# Autodesk Inventor assembly: ARM1
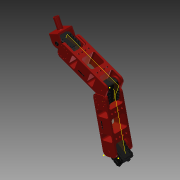
[picture p0: Inventor's stored thumbnail of the model, 180x180]
Saved by Autodesk Inventor 2015 (Build 190159000, 159)
## iProperties
Created: 2016-12-02
Part Number: ARM1
Document SubType Name: Assembly
Designer: Rudge-Top
Author: Rudge-Top
## Documents named in this file (4)
- C:\Users\Rudge-Top\Documents\RoboticArm\Inventor 2015\ARM1.iam
- C:\Users\Rudge-Top\Documents\RoboticArm\Inventor 2015\150mm Link.ipt
- C:\Users\Rudge-Top\Documents\RoboticArm\Inventor 2015\AX12.iam
- C:\Users\Rudge-Top\Documents\RoboticArm\Inventor 2015\Pen.ipt
## Components (6 placed, 3 different names)
1. 150mm Link:1 — Insert:1, Insert:2
2. AX12:1 [sub-assembly] — Insert:1
3. 150mm Link:2 — Insert:3, Insert:4
4. AX12:2 [sub-assembly] — Insert:2, Insert:3
5. Pen:1 — Insert:5
6. AX12:3 [sub-assembly] — Insert:4, Insert:5
## Relationships (5: Insert 5)
- Insert:1: 150mm Link:1 ↔ AX12:1
- Insert:2: 150mm Link:1 ↔ AX12:2
- Insert:3: 150mm Link:2 ↔ AX12:2
- Insert:4: 150mm Link:2 ↔ AX12:3
- Insert:5: Pen:1 ↔ AX12:3
